# Autodesk Inventor assembly: ADF4360-Enclosure
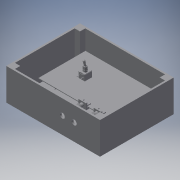
[picture p0: Inventor's stored thumbnail of the model, 180x180]
Saved by Autodesk Inventor 2018 (Build 220112000, 112)
## iProperties
Created: 2018-04-28
Part Number: ADF4360-Enclosure
Document SubType Name: Assembly
Designer: bbramman
Author: bbramman
## Documents named in this file (4)
- C:\Users\bbramman\OneDrive\Documents\Trapped Ion Research (Grad)\Electronics\pll-evalboard-synthesizer\Box CAD\ADF4360-Enclosure.iam
- C:\Users\bbramman\OneDrive\Documents\Trapped Ion Research (Grad)\Electronics\pll-evalboard-synthesizer\Box CAD\546-1590BBS-ADF4360-9.ipt
- C:\Users\bbramman\OneDrive\Documents\Trapped Ion Research (Grad)\Electronics\pll-evalboard-synthesizer\Box CAD\Power-Reg.iam
- C:\Users\bbramman\OneDrive\Documents\Trapped Ion Research (Grad)\Electronics\pll-evalboard-synthesizer\Box CAD\EV-ADF4360.iam
## Components (3 placed, 3 different names)
1. 546-1590BBS-ADF4360-9:1 — Insert:1
2. Power-Reg:1 [sub-assembly] — Insert:1
3. EV-ADF4360:1 [sub-assembly]
## Relationships (1: Insert 1)
- Insert:1 (6.35 mm): 546-1590BBS-ADF4360-9:1 ↔ Power-Reg:1
